# Autodesk Inventor assembly: Пандус
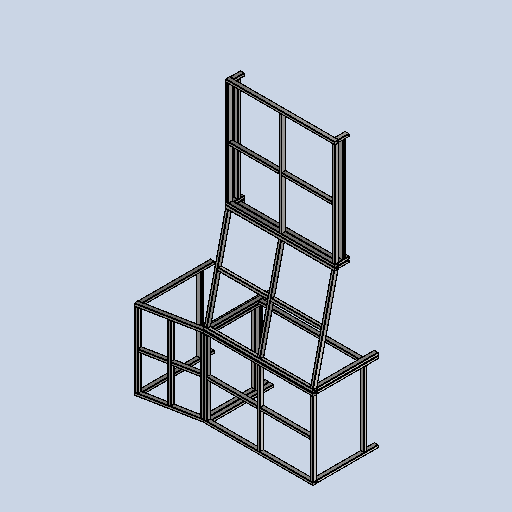
[picture p0: Inventor's stored thumbnail of the model, 512x512]
Saved by Autodesk Inventor 2025 (Build 290162010, 162A)
## iProperties
Created: 2024-09-18
Part Number: Пандус
Document SubType Name: Assembly
Designer: pokla
Author: pokla
## Documents named in this file (10)
- C:\Users\pokla\Documents\Inventor\BSH_Beshkino_bio_tank\Пандус.iam
- C:\Users\pokla\Documents\Inventor\BSH_Beshkino_bio_tank\Тумба 2.iam
- C:\Users\pokla\Documents\Inventor\BSH_Beshkino_bio_tank\Ноги тумба 2.iam
- C:\Users\pokla\Documents\Inventor\BSH_Beshkino_bio_tank\Тумба 4.iam
- C:\Users\pokla\Documents\Inventor\BSH_Beshkino_bio_tank\Ноги тумба 4.iam
- C:\Users\pokla\Documents\Inventor\BSH_Beshkino_bio_tank\Тумба 3.iam
- C:\Users\pokla\Documents\Inventor\BSH_Beshkino_bio_tank\Нога тумба 3.1.iam
- C:\Users\pokla\Documents\Inventor\BSH_Beshkino_bio_tank\Нога тумба 3.2.iam
- C:\Users\pokla\Documents\Inventor\BSH_Beshkino_bio_tank\Тумба 1.iam
- C:\Users\pokla\Documents\Inventor\BSH_Beshkino_bio_tank\Ноги тумба 1.iam
## Components (12 placed, 9 different names)
1. Тумба 2:1 [sub-assembly]
2. Ноги тумба 2:1 [sub-assembly]
3. Ноги тумба 2:2 [sub-assembly]
4. Тумба 4:1 [sub-assembly]
5. Ноги тумба 4:1 [sub-assembly]
6. Ноги тумба 4:2 [sub-assembly]
7. Тумба 3:1 [sub-assembly]
8. Нога тумба 3.1:1 [sub-assembly]
9. Нога тумба 3.2:1 [sub-assembly]
10. Тумба 1:1 [sub-assembly]
11. Ноги тумба 2:3 [sub-assembly]
12. Ноги тумба 1:1 [sub-assembly]
## Relationships (20: WeldJoint 7, Tangent 6, Flush 5, Mate 2)
- [WeldJoint]: Тумба 2:1 ↔ Ноги тумба 2:1
- [WeldJoint]: Тумба 2:1 ↔ Ноги тумба 2:2
- [WeldJoint]: Тумба 4:1 ↔ Ноги тумба 4:1
- [WeldJoint]: Тумба 4:1 ↔ Ноги тумба 4:2
- [WeldJoint]: Ноги тумба 2:1 ↔ Нога тумба 3.1:1
- [WeldJoint]: Ноги тумба 4:1 ↔ Нога тумба 3.2:1
- [Flush]: Тумба 2:1 ↔ Тумба 4:1
- [Tangent]: Тумба 3:1 ↔ Нога тумба 3.2:1
- [Tangent]: Тумба 3:1 ↔ Нога тумба 3.1:1
- [Flush]: Тумба 2:1 ↔ Тумба 3:1
- [Tangent]: Тумба 4:1 ↔ Тумба 3:1
- [Tangent]: Тумба 2:1 ↔ Тумба 3:1
- [WeldJoint]: Ноги тумба 2:2 ↔ Ноги тумба 2:3
- [Flush]: Ноги тумба 2:2 ↔ Ноги тумба 1:1
- [Flush]: Ноги тумба 2:3 ↔ Ноги тумба 1:1
- [Flush]: Тумба 1:1 ↔ Ноги тумба 2:3
- [Mate] (691 mm): Ноги тумба 2:3 ↔ Ноги тумба 1:1
- [Tangent]: Тумба 1:1 ↔ Ноги тумба 2:3
- [Tangent]: Тумба 1:1 ↔ Ноги тумба 1:1
- [Mate]: Тумба 1:1 ↔ Ноги тумба 1:1
